# Autodesk Inventor assembly: AssemblyGefreesdBasev2
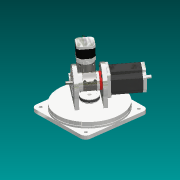
[picture p0: Inventor's stored thumbnail of the model, 180x180]
Saved by Autodesk Inventor 2020.3 (Build 243373000, 373)
## iProperties
Created: 2020-05-18
Part Number: AssemblyGefreesdBasev2
Document SubType Name: Assembly
Designer: Svend
Author: Svend
## Documents named in this file (22)
- C:\Users\Svend\OneDrive\Documents\GitHub\BeerMinder\3D-model\Base (Axis 1)\gefreesd\AssemblyGefreesdBasev2.iam
- C:\Users\Svend\OneDrive\Documents\GitHub\BeerMinder\3D-model\subAssembly\Nema17MetGearbox.iam
- C:\Users\Svend\OneDrive\Documents\GitHub\BeerMinder\3D-model\gearbox\afstandsplaatje.ipt
- C:\Users\Svend\OneDrive\Documents\GitHub\BeerMinder\3D-model\bearings\Ball Bearing 608ZZ.ipt
- C:\Users\Svend\OneDrive\Documents\GitHub\BeerMinder\3D-model\pulleys\GT2 Timing Pulley 20T - 8mm as.ipt
- C:\Users\Svend\OneDrive\Documents\GitHub\BeerMinder\3D-model\pulleys\GT2 Timing Pulley 60T - 8mm as.ipt
- C:\Users\Svend\OneDrive\Documents\GitHub\BeerMinder\3D-model\pulleys\Tandriem20naar60T.ipt
- C:\Users\Svend\OneDrive\Documents\GitHub\BeerMinder\3D-model\Base (Axis 1)\AsBase.ipt
- C:\Users\Svend\OneDrive\Documents\GitHub\BeerMinder\3D-model\subAssembly\Nema23MetGearbox.iam
- C:\Users\Svend\OneDrive\Documents\GitHub\BeerMinder\3D-model\Base (Axis 1)\gefreesd\base bovenkant v2.ipt
- C:\Users\Svend\OneDrive\Documents\GitHub\BeerMinder\3D-model\bearings\51110 Groefkogellager - 70 mm.iam
- C:\Users\Svend\OneDrive\Documents\GitHub\BeerMinder\3D-model\Base (Axis 1)\gefreesd\motorFrame.ipt
- C:\Users\Svend\OneDrive\Documents\GitHub\BeerMinder\3D-model\Base (Axis 1)\gefreesd\base onderkant.ipt
- C:\Users\Svend\OneDrive\Documents\GitHub\BeerMinder\3D-model\Base (Axis 1)\gefreesd\gearboxframv2.ipt
- C:\Users\Svend\OneDrive\Documents\Inventor\Content Center Files\R2020\en-US\ISO 7380-1\ISO 7380-1 - M4 x 12.ipt
- C:\Users\Svend\OneDrive\Documents\Inventor\Content Center Files\R2020\en-US\ISO 7380-1\ISO 7380-1 - M4 x 20.ipt
- C:\Users\Svend\OneDrive\Documents\GitHub\BeerMinder\3D-model\bearings\slewbearing\Slew Bearing v2 v18.iam
- C:\Users\Svend\OneDrive\Documents\Inventor\Content Center Files\R2020\en-US\ISO 7380-1\ISO 7380-1 - M3 x 10.ipt
- C:\Users\Svend\OneDrive\Documents\Inventor\Content Center Files\R2020\en-US\ISO 10642(1)\ISO 10642 - M4x16.ipt
- C:\Users\Svend\OneDrive\Documents\Inventor\Content Center Files\R2020\en-US\ISO 4035(2)\ISO 4035 - M3 - ISO.ipt
- C:\Users\Svend\OneDrive\Documents\Inventor\Content Center Files\R2020\en-US\ISO 10642(1)\ISO 10642 - M3x16.ipt
- C:\Users\Svend\OneDrive\Documents\GitHub\BeerMinder\3D-model\axis4\asmountAs4.ipt
## Components (54 placed, 21 different names)
1. base bovenkant v2:1 — Mate:20, Mate:7, Flush:5, Mate:46, Mate:60, Mate:63, Mate:121, Flush:118, Mate:196, Mate:197, Mate:198, Mate:199, Mate:200, Mate:201, Mate:202, Mate:203
2. Nema17MetGearbox:1 [sub-assembly] — Mate:20, Mate:52, Mate:56, Mate:58, Mate:59, Flush:6, Flush:12, Mate:121
3. Ball Bearing 608ZZ:1 — Mate:7, Mate:17, Flush:5, Mate:51
4. GT2 Timing Pulley 20T - 8mm as:1 — Mate:52, Mate:53, Mate:54, Flush:6
5. GT2 Timing Pulley 60T - 8mm as:1 — Mate:14, Mate:40, Mate:51, Mate:55, Flush:15
6. Tandriem20naar60T:1 — Mate:14, Mate:53, Mate:54, Mate:55, Flush:118
7. AsBase:1 — Mate:17, Mate:40, Mate:45, Mate:61, Flush:15, Mate:67, Mate:210
8. Nema23MetGearbox:1 [sub-assembly] — Mate:60, Mate:61, Flush:10, Flush:11, Mate:62, Mate:64, Flush:16, Flush:17, Mate:72, Mate:124, Mate:122
9. 51110 Groefkogellager - 70 mm:1 [sub-assembly] — Mate:45, Mate:46, Mate:71
10. afstandsplaatje:1 — Mate:56, Mate:58, Mate:59, Mate:90, Mate:91, Mate:92, Mate:93, Insert:1, Insert:2, Insert:3, Insert:4, Insert:5, Insert:6, Insert:7, Insert:8
11. motorFrame:1 — Flush:10, Flush:11, Mate:62, Mate:63, Mate:64, Flush:12, Mate:88, Mate:89, Mate:94, Mate:95, Mate:96, Mate:97, Mate:98, Mate:99, Mate:100, Mate:101
12. base onderkant:1 — Mate:67, Mate:71, Mate:138, Flush:121, Mate:139, Mate:211, Mate:212, Mate:213, Mate:214, Mate:215
13. gearboxframv2:1 — Flush:16, Flush:17, Mate:72, Mate:86, Mate:87, Mate:122, Mate:125, Mate:195
14. Slew Bearing v2 v18:1 [sub-assembly] — Mate:124, Mate:125, Mate:195, Insert:9, Insert:10, Insert:11, Insert:12, Insert:13, Insert:14, Insert:15, Insert:16, Mate:206, Mate:207, Mate:208, Mate:209
15. asmountAs4:1 — Mate:210, Mate:211, Mate:215
16. ISO 10642 M4x16:9 — Mate:212
17. ISO 10642 M4x16:10 — Mate:213
18. ISO 10642 M4x16:11 — Mate:214
19. ISO 7380-1 M4 x 12:1 — Mate:89, Mate:90
20. ISO 7380-1 M4 x 12:2 — Mate:88, Mate:91
21. ISO 7380-1 M4 x 12:3 — Mate:87, Mate:93
22. ISO 7380-1 M4 x 12:4 — Mate:86, Mate:92
23. ISO 7380-1 M4 x 20:1 — Mate:94, Mate:100
24. ISO 7380-1 M4 x 20:2 — Mate:95, Mate:99
25. ISO 7380-1 M4 x 20:4 — Mate:97, Mate:98
26. ISO 7380-1 M4 x 20:3 — Mate:96, Mate:101
27. ISO 4035 M3:1 — Insert:9
28. ISO 4035 M3:2 — Insert:10
29. ISO 4035 M3:3 — Insert:11
30. ISO 4035 M3:4 — Insert:12
31. ISO 4035 M3:5 — Insert:13
32. ISO 4035 M3:6 — Insert:14
33. ISO 4035 M3:7 — Insert:15
34. ISO 4035 M3:8 — Insert:16
35. ISO 10642 M3x16:1 — Mate:206
36. ISO 10642 M3x16:2 — Mate:207
37. ISO 10642 M3x16:3 — Mate:208
38. ISO 10642 M3x16:4 — Mate:209
39. ISO 10642 M4x16:1 — Mate:196
40. ISO 10642 M4x16:2 — Mate:197
41. ISO 10642 M4x16:3 — Mate:198
42. ISO 10642 M4x16:4 — Mate:199
43. ISO 10642 M4x16:5 — Mate:200
44. ISO 10642 M4x16:6 — Mate:201
45. ISO 10642 M4x16:7 — Mate:202
46. ISO 10642 M4x16:8 — Mate:203
47. ISO 7380-1 M3 x 10:1 — Insert:1
48. ISO 7380-1 M3 x 10:2 — Insert:2
49. ISO 7380-1 M3 x 10:3 — Insert:3
50. ISO 7380-1 M3 x 10:4 — Insert:4
51. ISO 7380-1 M3 x 10:5 — Insert:5
52. ISO 7380-1 M3 x 10:6 — Insert:6
53. ISO 7380-1 M3 x 10:7 — Insert:7
54. ISO 7380-1 M3 x 10:8 — Insert:8
## Relationships (90: Mate 64, Insert 16, Flush 10)
- Mate:20: base bovenkant v2:1 ↔ Nema17MetGearbox:1
- Mate:7: base bovenkant v2:1 ↔ Ball Bearing 608ZZ:1
- Mate:14: GT2 Timing Pulley 60T - 8mm as:1 ↔ Tandriem20naar60T:1
- Mate:17: Ball Bearing 608ZZ:1 ↔ AsBase:1
- Mate:40: GT2 Timing Pulley 60T - 8mm as:1 ↔ AsBase:1
- Flush:5: base bovenkant v2:1 ↔ Ball Bearing 608ZZ:1
- Mate:45: AsBase:1 ↔ 51110 Groefkogellager - 70 mm:1
- Mate:46: base bovenkant v2:1 ↔ 51110 Groefkogellager - 70 mm:1
- Mate:51: Ball Bearing 608ZZ:1 ↔ GT2 Timing Pulley 60T - 8mm as:1
- Mate:52: Nema17MetGearbox:1 ↔ GT2 Timing Pulley 20T - 8mm as:1
- Mate:53 (0.5 mm): GT2 Timing Pulley 20T - 8mm as:1 ↔ Tandriem20naar60T:1
- Mate:54: GT2 Timing Pulley 20T - 8mm as:1 ↔ Tandriem20naar60T:1
- Mate:55 (0.5 mm): GT2 Timing Pulley 60T - 8mm as:1 ↔ Tandriem20naar60T:1
- Mate:56: Nema17MetGearbox:1 ↔ afstandsplaatje:1
- Mate:58: Nema17MetGearbox:1 ↔ afstandsplaatje:1
- Mate:59: Nema17MetGearbox:1 ↔ afstandsplaatje:1
- Flush:6: Nema17MetGearbox:1 ↔ GT2 Timing Pulley 20T - 8mm as:1
- Mate:60 (20 mm): base bovenkant v2:1 ↔ Nema23MetGearbox:1
- Mate:61 (-29.76 mm): AsBase:1 ↔ Nema23MetGearbox:1
- Flush:10: Nema23MetGearbox:1 ↔ motorFrame:1
- Flush:11: Nema23MetGearbox:1 ↔ motorFrame:1
- Mate:62: Nema23MetGearbox:1 ↔ motorFrame:1
- Mate:63: base bovenkant v2:1 ↔ motorFrame:1
- Mate:64: Nema23MetGearbox:1 ↔ motorFrame:1
- Flush:12 (-26.25 mm): Nema17MetGearbox:1 ↔ motorFrame:1
- Flush:15: GT2 Timing Pulley 60T - 8mm as:1 ↔ AsBase:1
- Mate:67: AsBase:1 ↔ base onderkant:1
- Flush:16: Nema23MetGearbox:1 ↔ gearboxframv2:1
- Flush:17: Nema23MetGearbox:1 ↔ gearboxframv2:1
- Mate:71: 51110 Groefkogellager - 70 mm:1 ↔ base onderkant:1
- Mate:72: Nema23MetGearbox:1 ↔ gearboxframv2:1
- Mate:86: gearboxframv2:1 ↔ ISO 7380-1 M4 x 12:4
- Mate:87: gearboxframv2:1 ↔ ISO 7380-1 M4 x 12:3
- Mate:88: motorFrame:1 ↔ ISO 7380-1 M4 x 12:2
- Mate:89: motorFrame:1 ↔ ISO 7380-1 M4 x 12:1
- Mate:90: afstandsplaatje:1 ↔ ISO 7380-1 M4 x 12:1
- Mate:91: afstandsplaatje:1 ↔ ISO 7380-1 M4 x 12:2
- Mate:92: afstandsplaatje:1 ↔ ISO 7380-1 M4 x 12:4
- Mate:93: afstandsplaatje:1 ↔ ISO 7380-1 M4 x 12:3
- Mate:94: motorFrame:1 ↔ ISO 7380-1 M4 x 20:1
- Mate:95: motorFrame:1 ↔ ISO 7380-1 M4 x 20:2
- Mate:96: motorFrame:1 ↔ ISO 7380-1 M4 x 20:3
- Mate:97: motorFrame:1 ↔ ISO 7380-1 M4 x 20:4
- Mate:98: motorFrame:1 ↔ ISO 7380-1 M4 x 20:4
- Mate:99: motorFrame:1 ↔ ISO 7380-1 M4 x 20:2
- Mate:100: motorFrame:1 ↔ ISO 7380-1 M4 x 20:1
- Mate:101: motorFrame:1 ↔ ISO 7380-1 M4 x 20:3
- Mate:121: base bovenkant v2:1 ↔ Nema17MetGearbox:1
- Flush:118: base bovenkant v2:1 ↔ Tandriem20naar60T:1
- Mate:122: Nema23MetGearbox:1 ↔ gearboxframv2:1
- Mate:124: Nema23MetGearbox:1 ↔ Slew Bearing v2 v18:1
- Mate:125: gearboxframv2:1 ↔ Slew Bearing v2 v18:1
- Mate:138: base onderkant:1
- Flush:121: base onderkant:1
- Mate:139: base onderkant:1
- Mate:195: gearboxframv2:1 ↔ Slew Bearing v2 v18:1
- Insert:1: afstandsplaatje:1 ↔ ISO 7380-1 M3 x 10:1
- Insert:2: afstandsplaatje:1 ↔ ISO 7380-1 M3 x 10:2
- Insert:3: afstandsplaatje:1 ↔ ISO 7380-1 M3 x 10:3
- Insert:4: afstandsplaatje:1 ↔ ISO 7380-1 M3 x 10:4
- Insert:5: afstandsplaatje:1 ↔ ISO 7380-1 M3 x 10:5
- Insert:6: afstandsplaatje:1 ↔ ISO 7380-1 M3 x 10:6
- Insert:7: afstandsplaatje:1 ↔ ISO 7380-1 M3 x 10:7
- Insert:8: afstandsplaatje:1 ↔ ISO 7380-1 M3 x 10:8
- Mate:196: base bovenkant v2:1 ↔ ISO 10642 M4x16:1
- Mate:197: base bovenkant v2:1 ↔ ISO 10642 M4x16:2
- Mate:198: base bovenkant v2:1 ↔ ISO 10642 M4x16:3
- Mate:199: base bovenkant v2:1 ↔ ISO 10642 M4x16:4
- Mate:200: base bovenkant v2:1 ↔ ISO 10642 M4x16:5
- Mate:201: base bovenkant v2:1 ↔ ISO 10642 M4x16:6
- Mate:202: base bovenkant v2:1 ↔ ISO 10642 M4x16:7
- Mate:203: base bovenkant v2:1 ↔ ISO 10642 M4x16:8
- Insert:9: Slew Bearing v2 v18:1 ↔ ISO 4035 M3:1
- Insert:10: Slew Bearing v2 v18:1 ↔ ISO 4035 M3:2
- Insert:11: Slew Bearing v2 v18:1 ↔ ISO 4035 M3:3
- Insert:12: Slew Bearing v2 v18:1 ↔ ISO 4035 M3:4
- Insert:13: Slew Bearing v2 v18:1 ↔ ISO 4035 M3:5
- Insert:14: Slew Bearing v2 v18:1 ↔ ISO 4035 M3:6
- Insert:15: Slew Bearing v2 v18:1 ↔ ISO 4035 M3:7
- Insert:16: Slew Bearing v2 v18:1 ↔ ISO 4035 M3:8
- Mate:206: Slew Bearing v2 v18:1 ↔ ISO 10642 M3x16:1
- Mate:207: Slew Bearing v2 v18:1 ↔ ISO 10642 M3x16:2
- Mate:208: Slew Bearing v2 v18:1 ↔ ISO 10642 M3x16:3
- Mate:209: Slew Bearing v2 v18:1 ↔ ISO 10642 M3x16:4
- Mate:210: AsBase:1 ↔ asmountAs4:1
- Mate:211: base onderkant:1 ↔ asmountAs4:1
- Mate:212: base onderkant:1 ↔ ISO 10642 M4x16:9
- Mate:213: base onderkant:1 ↔ ISO 10642 M4x16:10
- Mate:214: base onderkant:1 ↔ ISO 10642 M4x16:11
- Mate:215: base onderkant:1 ↔ asmountAs4:1
